# Autodesk Inventor assembly: A2017_T3_05
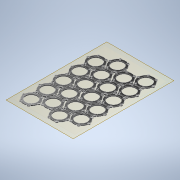
[picture p0: Inventor's stored thumbnail of the model, 180x180]
Saved by Autodesk Inventor 2022 (Build 260153000, 153)
## iProperties
Created: 2022-09-28
Part Number: A2017_T3_05
Document SubType Name: Assembly
Designer: Masato
Author: Masato
## Documents named in this file (3)
- C:\Users\6343y\ドキュメント\Inventor\SUSTAINA-OP\Cam\A2017_T3\A2017_T3_05.iam
- C:\Users\6343y\ドキュメント\Inventor\SUSTAINA-OP\Cam\DisposableBoard.ipt
- C:\Users\6343y\ドキュメント\Inventor\SUSTAINA-OP\UpperBody\Trunk\CrossRollerBearing\Outer_flange.ipt
## Components (21 placed, 2 different names)
1. DisposableBoard:1 — フラッシュ:1, フラッシュ:2, フラッシュ:3, フラッシュ:4, 正接:1, 正接:2, 正接:3
2. Outer_flange:1 — メイト:1, 正接:1, 正接:2, 正接:3, 角度:1, 角度:2, 正接:4
3. Outer_flange:2 — メイト:2, 角度:1, 角度:2, 正接:4
4. Outer_flange:3
5. Outer_flange:4
6. Outer_flange:5
7. Outer_flange:6
8. Outer_flange:7
9. Outer_flange:8
10. Outer_flange:9
11. Outer_flange:10
12. Outer_flange:11
13. Outer_flange:12
14. Outer_flange:13
15. Outer_flange:14
16. Outer_flange:15
17. Outer_flange:16
18. Outer_flange:17
19. Outer_flange:18
20. Outer_flange:19
21. Outer_flange:20
## Component patterns: (10 elements, first: Outer_flange:1 + Outer_flange:2)
## Relationships (12: Flush 4, Tangent 4, Mate 2, Angle 2)
- フラッシュ:1 [Flush]: DisposableBoard:1
- フラッシュ:2 [Flush]: DisposableBoard:1
- フラッシュ:3 [Flush]: DisposableBoard:1
- フラッシュ:4 [Flush]: DisposableBoard:1
- メイト:1 [Mate]: Outer_flange:1
- 正接:1 [Tangent] (2.1 mm): DisposableBoard:1 ↔ Outer_flange:1
- 正接:2 [Tangent] (2.1 mm): DisposableBoard:1 ↔ Outer_flange:1
- 正接:3 [Tangent] (2.1 mm): DisposableBoard:1 ↔ Outer_flange:1
- メイト:2 [Mate]: Outer_flange:2
- 角度:1 [Angle] (0 deg): Outer_flange:1 ↔ Outer_flange:2
- 角度:2 [Angle] (0 deg): Outer_flange:1 ↔ Outer_flange:2
- 正接:4 [Tangent] (2.1 mm): Outer_flange:1 ↔ Outer_flange:2
